# Autodesk Inventor assembly: TotalAssembly
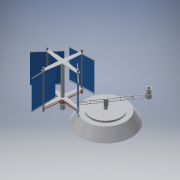
[picture p0: Inventor's stored thumbnail of the model, 180x180]
Saved by Autodesk Inventor 2018 (Build 220112000, 112)
## iProperties
Created: 2016-07-04
Part Number: TotalAssembly
Document SubType Name: Assembly
Designer: Tore Den Store
Author: Tore Den Store
## Documents named in this file (5)
- C:\Users\ToreDenStore\Documents\Inventor\Vertical axis wind turbine\TotalAssembly.iam
- C:\Users\ToreDenStore\Documents\Inventor\Vertical axis wind turbine\BaseAssembly.iam
- C:\Users\ToreDenStore\Documents\Inventor\Vertical axis wind turbine\WindPartCentral\Connecting gears.ipt
- C:\Users\ToreDenStore\Documents\Inventor\Vertical axis wind turbine\WindPartCentral\WindCentralbeam.ipt
- C:\Users\ToreDenStore\Documents\Inventor\Vertical axis wind turbine\1 of 4 part\SailBeam.iam
## Components (10 placed, 4 different names)
1. BaseAssembly:1 [sub-assembly] — Rotational:15, Rotation:1, Rotation:2, Rotation:3, Rotation:4
2. Connecting gears:1 — Rotational:14, Rotation:1
3. WindCentralbeam:1 — Rotational:5, Rotational:6, Rotational:8, Rotational:9, Rotational:10, Rotational:11, Rotational:13, Rotational:14, Rotational:15, Rotation:5, Rotation:6, Rotation:7, Rotation:8
4. SailBeam:1 [sub-assembly] — Rotational:5, Rotation:7
5. SailBeam:2 [sub-assembly] — Rotational:6, Rotation:6
6. Connecting gears:2 — Rotational:13, Rotation:2
7. Connecting gears:3 — Rotational:8, Rotation:3
8. Connecting gears:4 — Rotational:9, Rotation:4
9. SailBeam:3 [sub-assembly] — Rotational:10, Rotation:5
10. SailBeam:4 [sub-assembly] — Rotational:11, Rotation:8
## Relationships (17: RevoluteJoint 9, RelateRotation 8)
- Rotational:5 [RevoluteJoint]: WindCentralbeam:1 ↔ SailBeam:1
- Rotational:6 [RevoluteJoint]: WindCentralbeam:1 ↔ SailBeam:2
- Rotational:8 [RevoluteJoint]: WindCentralbeam:1 ↔ Connecting gears:3
- Rotational:9 [RevoluteJoint]: WindCentralbeam:1 ↔ Connecting gears:4
- Rotational:10 [RevoluteJoint]: WindCentralbeam:1 ↔ SailBeam:3
- Rotational:11 [RevoluteJoint]: WindCentralbeam:1 ↔ SailBeam:4
- Rotational:13 [RevoluteJoint]: WindCentralbeam:1 ↔ Connecting gears:2
- Rotational:14 [RevoluteJoint]: Connecting gears:1 ↔ WindCentralbeam:1
- Rotational:15 [RevoluteJoint]: BaseAssembly:1 ↔ WindCentralbeam:1
- Rotation:1 [RelateRotation] (0.8 ul): BaseAssembly:1 ↔ Connecting gears:1
- Rotation:2 [RelateRotation] (0.8 ul): BaseAssembly:1 ↔ Connecting gears:2
- Rotation:3 [RelateRotation] (0.8 ul): BaseAssembly:1 ↔ Connecting gears:3
- Rotation:4 [RelateRotation] (0.8 ul): BaseAssembly:1 ↔ Connecting gears:4
- Rotation:5 [RelateRotation] (2 ul): WindCentralbeam:1 ↔ SailBeam:3
- Rotation:6 [RelateRotation] (2 ul): WindCentralbeam:1 ↔ SailBeam:2
- Rotation:7 [RelateRotation] (2 ul): WindCentralbeam:1 ↔ SailBeam:1
- Rotation:8 [RelateRotation] (2 ul): WindCentralbeam:1 ↔ SailBeam:4
